# Autodesk Inventor assembly: Assembly1
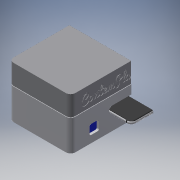
[picture p0: Inventor's stored thumbnail of the model, 180x180]
Saved by Autodesk Inventor 2019 (Build 230136000, 136)
## iProperties
Created: 2018-06-15
Part Number: Assembly1
Document SubType Name: Assembly
Designer: daniel
Author: daniel
## Documents named in this file (11)
- D:\googledrive\PCPS\TOP SECRET\Modelle\Assembly1.iam
- D:\googledrive\PCPS\TOP SECRET\Modelle\body.ipt
- D:\googledrive\PCPS\TOP SECRET\Modelle\arduino\arduino uno.iam
- D:\googledrive\PCPS\TOP SECRET\Modelle\iphone8plus\i8 plus.ipt
- D:\googledrive\PCPS\TOP SECRET\Modelle\divider.ipt
- D:\googledrive\PCPS\TOP SECRET\Modelle\button.ipt
- D:\googledrive\PCPS\TOP SECRET\Modelle\scharnier.ipt
- D:\googledrive\PCPS\TOP SECRET\Modelle\plate.ipt
- D:\googledrive\PCPS\TOP SECRET\Modelle\lcdsw.ipt
- D:\googledrive\PCPS\TOP SECRET\Modelle\oledlcd.ipt
- D:\googledrive\PCPS\TOP SECRET\Modelle\lid2.ipt
## Components (11 placed, 11 different names)
1. body:1 — Flush:1, Flush:2, Flush:3, Mate:1, Mate:2, Mate:3, Mate:4, Mate:5, Mate:6, Mate:9, Mate:13, Mate:14, Mate:15, Flush:10, Mate:16, Flush:11, Mate:17
2. arduino uno:1 [sub-assembly] — Flush:4, Flush:5, Flush:6, Mate:1, Flush:7, Mate:2
3. base shield [sub-assembly] — Flush:4, Flush:5, Flush:6
4. i8 plus:1 — Mate:3, Mate:9
5. divider:1 — Mate:4, Flush:9, Mate:5
6. button:1 — Mate:6
7. scharnier:1 — Insert:3, Insert:4, Mate:17
8. plate:1 — Insert:3, Insert:4
9. lcdsw:1
10. oledlcd:1 — Mate:13, Mate:14, Mate:15
11. lid2:1 — Flush:10, Mate:16, Flush:11
## Relationships (24: Mate 12, Flush 10, Insert 2)
- Flush:1: body:1
- Flush:2: body:1
- Flush:3: body:1
- Flush:4: arduino uno:1 ↔ base shield
- Flush:5: arduino uno:1 ↔ base shield
- Flush:6: arduino uno:1 ↔ base shield
- Mate:1: body:1 ↔ arduino uno:1
- Flush:7 (40 mm): arduino uno:1
- Mate:2: body:1 ↔ arduino uno:1
- Mate:3 (5 mm): body:1 ↔ i8 plus:1
- Mate:4: body:1 ↔ divider:1
- Flush:9: divider:1
- Mate:5 (0.5 mm): body:1 ↔ divider:1
- Mate:6: body:1 ↔ button:1
- Insert:3: scharnier:1 ↔ plate:1
- Insert:4: scharnier:1 ↔ plate:1
- Mate:9 (1 mm): body:1 ↔ i8 plus:1
- Mate:13: body:1 ↔ oledlcd:1
- Mate:14: body:1 ↔ oledlcd:1
- Mate:15: body:1 ↔ oledlcd:1
- Flush:10: body:1 ↔ lid2:1
- Mate:16 (1 mm): body:1 ↔ lid2:1
- Flush:11: body:1 ↔ lid2:1
- Mate:17 (3 mm): body:1 ↔ scharnier:1
